# Autodesk Inventor assembly: MG-Kickerboard Winkel
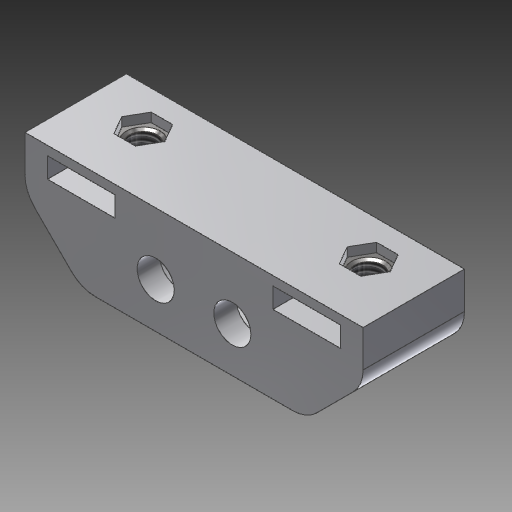
[picture p0: Inventor's stored thumbnail of the model, 512x512]
Saved by Autodesk Inventor 2019.4 (Build 234330000, 330)
## iProperties
Part Number: MG-Kickerboard Winkel
Material: Generisch
Document SubType Name: Assembly
Designer: rYan
Mass: 1.24098 g
Surface Area: 19.6577 cm^2
Volume: 1.56289 cm^3
Density: 0.794029 g/cm^3
Author: rYan
## Documents named in this file (3)
- D:\TIGERsGIT\Hardware\mechanik\2020\Inventor\Robot\Kicker\MG-Kickerboard Winkel.iam
- D:\TIGERsGIT\Hardware\mechanik\2020\Inventor\Robot\Kicker\Kickerboard Winkel.ipt
- D:\TIGERsGIT\Hardware\mechanik\2020\Inventor\Inhaltscenter\de-DE\DIN 562\DIN 562 - M3 x 5,5.ipt
## Components (3 placed, 2 different names)
1. Kickerboard Winkel:1 — Fluchtend:1, Fluchtend:2, Fluchtend:3, Passend:2, Passend:6, Passend:7, Passend:8, Passend:9, Passend:10
2. DIN 562 M3:2 — Passend:2, Passend:7, Passend:8
3. DIN 562 M3:3 — Passend:6, Passend:9, Passend:10
## Relationships (9: Mate 6, Flush 3)
- Fluchtend:1 [Flush]: Kickerboard Winkel:1
- Fluchtend:2 [Flush]: Kickerboard Winkel:1
- Fluchtend:3 [Flush]: Kickerboard Winkel:1
- Passend:2 [Mate] (0.1 mm): Kickerboard Winkel:1 ↔ DIN 562 M3:2
- Passend:6 [Mate] (0.1 mm): Kickerboard Winkel:1 ↔ DIN 562 M3:3
- Passend:7 [Mate] (0.25 mm): Kickerboard Winkel:1 ↔ DIN 562 M3:2
- Passend:8 [Mate] (0.25 mm): Kickerboard Winkel:1 ↔ DIN 562 M3:2
- Passend:9 [Mate] (0.25 mm): Kickerboard Winkel:1 ↔ DIN 562 M3:3
- Passend:10 [Mate] (0.25 mm): Kickerboard Winkel:1 ↔ DIN 562 M3:3
